# Autodesk Inventor assembly: Matchboxscope_v0
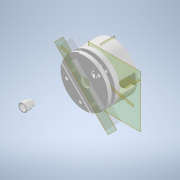
[picture p0: Inventor's stored thumbnail of the model, 180x180]
Saved by Autodesk Inventor 2022 (Build 260153000, 153)
## iProperties
Created: 2022-03-21
Part Number: Matchboxscope_v0
Document SubType Name: Assembly
Designer: Prakash Lab
Author: Prakash Lab
## Documents named in this file (8)
- C:\Users\PrakashLab\Documents\Matchboxscope\INVENTOR\Matchboxscope_v0.iam
- C:\Users\PrakashLab\Documents\Matchboxscope\INVENTOR\Matchboxscope_bottom_v0.ipt
- C:\Users\PrakashLab\Documents\Matchboxscope\INVENTOR\Matchboxscope_middle2_v1.ipt
- C:\Users\PrakashLab\Documents\Matchboxscope\INVENTOR\00_ESP3-CAM.iam
- C:\Users\PrakashLab\Documents\Matchboxscope\INVENTOR\camera for ESP32 v1.iam
- C:\Users\PrakashLab\Documents\Matchboxscope\INVENTOR\00_chip.ipt
- C:\Users\PrakashLab\Documents\Matchboxscope\INVENTOR\Matchboxscope_sample_v0.ipt
- C:\Users\PrakashLab\Documents\Matchboxscope\INVENTOR\Matchboxscope_lenstube_v0.ipt
## Components (8 placed, 7 different names)
1. Matchboxscope_bottom_v0:1 — Mate:1, Flush:1, Mate:2, Angle:1, Insert:1
2. camera for ESP32 v1:1 [sub-assembly]
3. 00_chip:1 — Angle:1
4. Matchboxscope_sample_v0:1 — Insert:2
5. Matchboxscope_middle2_v1:1 — Insert:1, Insert:2
6. Matchboxscope_lenstube_v0:1
7. 00_ESP3-CAM:1 [sub-assembly] — Mate:1, Flush:1
8. 00_ESP3-CAM:3 [sub-assembly] — Mate:2
## Component patterns: (2 elements, first: 00_ESP3-CAM:1)
## Relationships (6: Mate 2, Insert 2, Flush 1, Angle 1)
- Mate:1: Matchboxscope_bottom_v0:1 ↔ 00_ESP3-CAM:1
- Flush:1: Matchboxscope_bottom_v0:1 ↔ 00_ESP3-CAM:1
- Mate:2 (1 mm): Matchboxscope_bottom_v0:1 ↔ 00_ESP3-CAM:3
- Angle:1 (135 deg): Matchboxscope_bottom_v0:1 ↔ 00_chip:1
- Insert:1: Matchboxscope_bottom_v0:1 ↔ Matchboxscope_middle2_v1:1
- Insert:2 (4 mm): Matchboxscope_sample_v0:1 ↔ Matchboxscope_middle2_v1:1
